# Autodesk Inventor assembly: motor3+fan
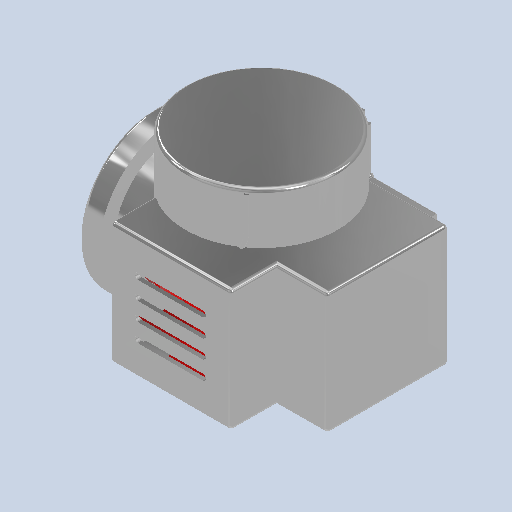
[picture p0: Inventor's stored thumbnail of the model, 512x512]
Saved by Autodesk Inventor 2023 (Build 270158000, 158)
## iProperties
Created: 2022-11-07
Part Number: motor3+fan
Document SubType Name: Assembly
Designer: willy
Author: willy
## Documents named in this file (3)
- C:\Users\willy\Documents\SPOT\motor3+fan.iam
- C:\Users\willy\Documents\SPOT\motor3+fan.ipt
- C:\Users\willy\Documents\SPOT\fan.ipt
## Components (2 placed, 2 different names)
1. motor3+fan:1 — 삽입:1
2. fan:1 — 삽입:1
## Relationships (1: Insert 1)
- 삽입:1 [Insert]: motor3+fan:1 ↔ fan:1
